# Autodesk Inventor assembly: miniSumo
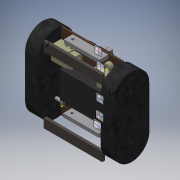
[picture p0: Inventor's stored thumbnail of the model, 180x180]
Saved by Autodesk Inventor 2016 (Build 200138000, 138)
## iProperties
Created: 2015-11-09
Part Number: miniSumo
Material: Ogólny
Document SubType Name: Assembly
Designer: Mrianura
Author: Mrianura
## Documents named in this file (11)
- C:\Users\Mrianura\Documents\Inventor\katorga\miniSumo.iam
- C:\Users\Mrianura\Documents\Inventor\katorga\gasienice.ipt
- C:\Users\Mrianura\Documents\Inventor\katorga\SharpIRsensor.ipt
- C:\Users\Mrianura\Documents\Inventor\katorga\plolu z obudowa.iam
- C:\Users\Mrianura\Documents\Inventor\katorga\plytka2.ipt
- C:\Users\Mrianura\Documents\Inventor\katorga\Zespół2.iam
- C:\Users\Mrianura\Documents\Inventor\katorga\li-pol.ipt
- C:\Users\Mrianura\Documents\Inventor\katorga\zderzaki.ipt
- C:\Users\Mrianura\Documents\Inventor\katorga\sfth7773.ipt
- C:\Users\Mrianura\Documents\Inventor\katorga\KTIR.ipt
- C:\Users\Mrianura\Documents\Inventor\katorga\mocowanie_luzem.ipt
## Components (15 placed, 10 different names)
1. gasienice:1 — Zestawiający:1, Styczny:1, Zestawiający:6, Wstaw:2
2. gasienice:2 — Zestawiający:1, Zestawiający:7, Wstaw:1
3. SharpIRsensor:1 — Zestawiający:4, Zestawiający:8
4. plolu z obudowa:1 [sub-assembly] — Zestawiający:7
5. plolu z obudowa:2 [sub-assembly] — Zestawiający:6
6. plytka2:1 — Zestawiający:4, Zestawiający:5, Zestawiający:9, Zestawiający:10, Zestawiający:13, Zestawiający:14
7. Zespół2:1 [sub-assembly]
8. li-pol:1 — Zestawiający:5
9. zderzaki:1 — Styczny:1, Zestawiający:11, Zestawiający:12
10. sfth7773:1 — Zestawiający:8, Zestawiający:10
11. sfth7773:2 — Zestawiający:9
12. KTIR:1 — Zestawiający:12
13. KTIR:2 — Zestawiający:11
14. mocowanie_luzem:1 — Zestawiający:14, Wstaw:2
15. mocowanie_luzem:2 — Zestawiający:13, Wstaw:1
## Relationships (16: Mate 13, Insert 2, Tangent 1)
- Zestawiający:1 [Mate] (70 mm): gasienice:1 ↔ gasienice:2
- [Mate]: plytka2:1 ↔ Zespół2:1
- Zestawiający:4 [Mate]: SharpIRsensor:1 ↔ plytka2:1
- Zestawiający:5 [Mate]: plytka2:1 ↔ li-pol:1
- Styczny:1 [Tangent]: gasienice:1 ↔ zderzaki:1
- Zestawiający:6 [Mate]: gasienice:1 ↔ plolu z obudowa:2
- Zestawiający:7 [Mate]: gasienice:2 ↔ plolu z obudowa:1
- Zestawiający:8 [Mate]: SharpIRsensor:1 ↔ sfth7773:1
- Zestawiający:9 [Mate]: plytka2:1 ↔ sfth7773:2
- Zestawiający:10 [Mate]: plytka2:1 ↔ sfth7773:1
- Zestawiający:11 [Mate]: zderzaki:1 ↔ KTIR:2
- Zestawiający:12 [Mate]: zderzaki:1 ↔ KTIR:1
- Zestawiający:13 [Mate]: plytka2:1 ↔ mocowanie_luzem:2
- Wstaw:1 [Insert]: gasienice:2 ↔ mocowanie_luzem:2
- Zestawiający:14 [Mate]: plytka2:1 ↔ mocowanie_luzem:1
- Wstaw:2 [Insert]: gasienice:1 ↔ mocowanie_luzem:1
